# Autodesk Inventor assembly: Breaker
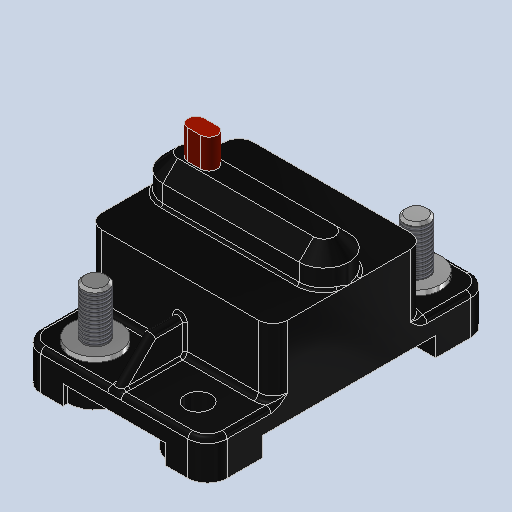
[picture p0: Inventor's stored thumbnail of the model, 512x512]
Saved by Autodesk Inventor 2023 (Build 270158000, 158)
## iProperties
Shininess: 64.0
Angle Display Precision: 2
Document Length Units: 11272
Document Angle Units: 11279
Document Time Units: 11290
Document Mass Units: 11286
Document Length Units Precision: 3
Document Angle Units Precision: 2
Created: 2004-01-20
Part Number: Breaker
Document SubType Name: Assembly
Designer: t8558es
Mass: 93.6381 g
Surface Area: 152.978 cm^2
Volume: 60.9774 cm^3
Density: 1.53562 g/cm^3
Density: 0.0
Volumn: 0.0
Area: 0.0
PropertySet Name: Model Information
Control State: 0
Master: False
Checked Out: False
Author: t8558es
## Documents named in this file (3)
- C:\Users\slick\OneDrive\Desktop\Crescendo_2024-CAD\2024 Robot\COMMON PARTS\ELECTRONICS\Breaker\Breaker.iam
- C:\Users\slick\OneDrive\Desktop\Crescendo_2024-CAD\2024 Robot\COMMON PARTS\ELECTRONICS\Breaker\Breaker Body.ipt
- C:\Users\slick\OneDrive\Desktop\Crescendo_2024-CAD\2024 Robot\COMMON PARTS\ELECTRONICS\Breaker\Breaker Post.ipt
## Components (3 placed, 2 different names)
1. Breaker Body:1 — Mate:1, Mate:2, Mate:3, Mate:4
2. Breaker Post:1 — Mate:1, Mate:2
3. Breaker Post:2 — Mate:3, Mate:4
## Relationships (4: Mate 4)
- Mate:1: Breaker Body:1 ↔ Breaker Post:1
- Mate:2: Breaker Body:1 ↔ Breaker Post:1
- Mate:3: Breaker Body:1 ↔ Breaker Post:2
- Mate:4: Breaker Body:1 ↔ Breaker Post:2
